# Autodesk Inventor assembly: servo_asm
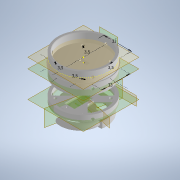
[picture p0: Inventor's stored thumbnail of the model, 180x180]
Saved by Autodesk Inventor 2020 (Build 240168000, 168)
## iProperties
Created: 2022-06-15
Part Number: servo_asm
Document SubType Name: Assembly
Designer: sp
Author: sp
## Documents named in this file (4)
- C:\Users\sp\Desktop\neu_Rocket\servo_asm.iam
- C:\Users\sp\Desktop\neu_Rocket\Servo_holder.ipt
- C:\Users\sp\Desktop\neu_Rocket\Verbindungsring.ipt
- C:\Users\sp\Desktop\neu_Rocket\Servo_Kupplung_V2.ipt
## Components (3 placed, 3 different names)
1. Servo_holder:1 — Einfügen:1, Passend:1, Einfügen:2
2. Verbindungsring:1 — Einfügen:1, Passend:1
3. Servo_Kupplung_V2:1 — Einfügen:2
## Relationships (3: Insert 2, Mate 1)
- Einfügen:1 [Insert] (20 mm): Servo_holder:1 ↔ Verbindungsring:1
- Passend:1 [Mate]: Servo_holder:1 ↔ Verbindungsring:1
- Einfügen:2 [Insert] (10 mm): Servo_holder:1 ↔ Servo_Kupplung_V2:1
